# Autodesk Inventor assembly: hand
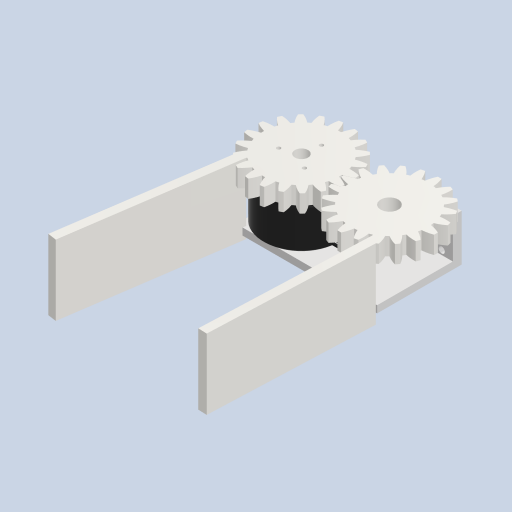
[picture p0: Inventor's stored thumbnail of the model, 512x512]
Saved by Autodesk Inventor 2023 (Build 270158000, 158)
## iProperties
Created: 2024-11-08
Part Number: hand
Document SubType Name: Assembly
Designer: kiyo
Author: kiyo
## Documents named in this file (7)
- D:\GitHub\inventor\syu-si\OfficeRobot\Manipulator\hand.iam
- D:\GitHub\inventor\OfficeRobot\ReadyMade\Steadywin\GIM3505-8.ipt
- D:\GitHub\inventor\OfficeRobot\Manipulator\hand_parts_1.ipt
- D:\GitHub\inventor\OfficeRobot\Manipulator\hand_parts_2.ipt
- D:\GitHub\inventor\OfficeRobot\Manipulator\gear_box.ipt
- D:\GitHub\inventor\OfficeRobot\ReadyMade\Screw\D3040-7130B.ipt
- D:\GitHub\inventor\OfficeRobot\ReadyMade\Screw\D4050-9120B.ipt
## Components (6 placed, 6 different names)
1. GIM3505-8:1 — 挿入:1, 挿入:2, 挿入:3
2. 平歯車1:1 — 挿入:1, フラッシュ:1
3. 平歯車2:1 — フラッシュ:1, 挿入:6
4. gear_box:1 — 挿入:2, 挿入:3, 挿入:7
5. D3040-7130B:1 — 挿入:5, 挿入:7
6. D4050-9120B:1 — 挿入:5, 挿入:6
## Relationships (7: Insert 6, Flush 1)
- 挿入:1 [Insert]: GIM3505-8:1 ↔ 平歯車1:1
- フラッシュ:1 [Flush]: 平歯車1:1 ↔ 平歯車2:1
- 挿入:2 [Insert]: GIM3505-8:1 ↔ gear_box:1
- 挿入:3 [Insert]: GIM3505-8:1 ↔ gear_box:1
- 挿入:5 [Insert]: D3040-7130B:1 ↔ D4050-9120B:1
- 挿入:6 [Insert]: 平歯車2:1 ↔ D4050-9120B:1
- 挿入:7 [Insert]: gear_box:1 ↔ D3040-7130B:1
